# Autodesk Inventor assembly: Robot Assembly MK2
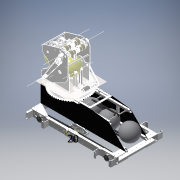
[picture p0: Inventor's stored thumbnail of the model, 180x180]
Saved by Autodesk Inventor 2019.4 (Build 234330000, 330)
## iProperties
Created: 2020-01-18
Part Number: Robot Assembly MK2
Document SubType Name: Assembly
Designer: Mark
Mass: 25008.8 g
Surface Area: 53804.7 cm^2
Volume: 25976.5 cm^3
Density: 0.96275 g/cm^3
Author: Mark
## Documents named in this file (4)
- C:\Users\Mark\Desktop\7738 Helion Engineering\7738-2020\Robot Assembly MK2.iam
- C:\Users\Mark\Desktop\7738 Helion Engineering\7738-2020\CAD\Drivebase.iam
- C:\Users\Mark\Desktop\7738 Helion Engineering\7738-2020\Upper Stage\Upper Stage.iam
- C:\Users\Mark\Desktop\7738 Helion Engineering\7738-2020\Robot V2\Turret Columb Assembly\Turret Columb Assembly.iam
## Components (3 placed, 3 different names)
1. Drivebase:1 [sub-assembly] — Mate:1, Flush:1, Flush:2
2. Upper Stage:1 [sub-assembly] — Mate:1, Flush:1, Flush:2, Mate:2, Mate:3
3. Turret Columb Assembly:1 [sub-assembly] — Mate:2, Mate:3
## Relationships (5: Mate 3, Flush 2)
- Mate:1: Drivebase:1 ↔ Upper Stage:1
- Flush:1: Drivebase:1 ↔ Upper Stage:1
- Flush:2: Drivebase:1 ↔ Upper Stage:1
- Mate:2: Upper Stage:1 ↔ Turret Columb Assembly:1
- Mate:3 (0.05 mm): Upper Stage:1 ↔ Turret Columb Assembly:1
